# Autodesk Inventor assembly: POM_T5_02
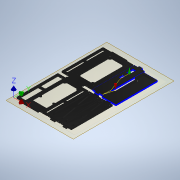
[picture p0: Inventor's stored thumbnail of the model, 180x180]
Saved by Autodesk Inventor 2020 (Build 240168000, 168)
## iProperties
Created: 2021-08-27
Part Number: POM_T5_02
Document SubType Name: Assembly
Designer: Masato
Author: Masato
## Documents named in this file (8)
- C:\Inventor\最新\OpenPlatform_ver3_0\Cam\POM_T5_02.iam
- C:\Inventor\最新\OpenPlatform_ver3_0\Cam\DisposableBoard.ipt
- C:\Inventor\最新\OpenPlatform_ver3_0\UpperBody\Cockpit\Cockpit_carrier_board_frame.ipt
- C:\Inventor\最新\OpenPlatform_ver3_0\UpperBody\Cockpit\Cockpit_circuit_board_frame.ipt
- C:\Inventor\最新\OpenPlatform_ver3_0\UpperBody\Cockpit\Cockpit_back_frame.ipt
- C:\Inventor\最新\OpenPlatform_ver3_0\UpperBody\Cockpit\Cockpit_battery_back_door.ipt
- C:\Inventor\最新\OpenPlatform_ver3_0\UpperBody\Cockpit\Cockpit_battery_bottom_frame.ipt
- C:\Inventor\最新\OpenPlatform_ver3_0\UpperBody\Cockpit\Cockpit_battery_front_frame.ipt
## Components (7 placed, 7 different names)
1. DisposableBoard:1 — メイト:2, メイト:1, フラッシュ:1, フラッシュ:2, メイト:4, メイト:6, メイト:7, メイト:8, メイト:9, フラッシュ:3, フラッシュ:4, フラッシュ:6, フラッシュ:7, メイト:17, フラッシュ:8
2. Cockpit_carrier_board_frame:1 — メイト:4, フラッシュ:3, フラッシュ:4, メイト:11, メイト:18
3. Cockpit_circuit_board_frame:1 — メイト:17, メイト:18, フラッシュ:8
4. Cockpit_back_frame:1 — メイト:9, メイト:12, メイト:16
5. Cockpit_battery_back_door:1 — メイト:8, メイト:15, メイト:16
6. Cockpit_battery_bottom_frame:1 — メイト:6, フラッシュ:6, メイト:11, メイト:12, メイト:14
7. Cockpit_battery_front_frame:1 — メイト:7, フラッシュ:7, メイト:14, メイト:15
## Relationships (21: Mate 14, Flush 7)
- メイト:2 [Mate]: DisposableBoard:1
- メイト:1 [Mate]: DisposableBoard:1
- フラッシュ:1 [Flush]: DisposableBoard:1
- フラッシュ:2 [Flush]: DisposableBoard:1
- メイト:4 [Mate]: DisposableBoard:1 ↔ Cockpit_carrier_board_frame:1
- メイト:6 [Mate]: DisposableBoard:1 ↔ Cockpit_battery_bottom_frame:1
- メイト:7 [Mate]: DisposableBoard:1 ↔ Cockpit_battery_front_frame:1
- メイト:8 [Mate]: DisposableBoard:1 ↔ Cockpit_battery_back_door:1
- メイト:9 [Mate]: DisposableBoard:1 ↔ Cockpit_back_frame:1
- フラッシュ:3 [Flush] (2.5 mm): DisposableBoard:1 ↔ Cockpit_carrier_board_frame:1
- フラッシュ:4 [Flush] (2.5 mm): DisposableBoard:1 ↔ Cockpit_carrier_board_frame:1
- フラッシュ:6 [Flush] (2.5 mm): DisposableBoard:1 ↔ Cockpit_battery_bottom_frame:1
- メイト:11 [Mate] (2.5 mm): Cockpit_carrier_board_frame:1 ↔ Cockpit_battery_bottom_frame:1
- メイト:12 [Mate] (2.5 mm): Cockpit_back_frame:1 ↔ Cockpit_battery_bottom_frame:1
- フラッシュ:7 [Flush] (2.5 mm): DisposableBoard:1 ↔ Cockpit_battery_front_frame:1
- メイト:14 [Mate] (2.5 mm): Cockpit_battery_bottom_frame:1 ↔ Cockpit_battery_front_frame:1
- メイト:15 [Mate] (2.5 mm): Cockpit_battery_back_door:1 ↔ Cockpit_battery_front_frame:1
- メイト:16 [Mate] (2.5 mm): Cockpit_back_frame:1 ↔ Cockpit_battery_back_door:1
- メイト:17 [Mate]: DisposableBoard:1 ↔ Cockpit_circuit_board_frame:1
- メイト:18 [Mate] (2.5 mm): Cockpit_carrier_board_frame:1 ↔ Cockpit_circuit_board_frame:1
- フラッシュ:8 [Flush] (2.5 mm): DisposableBoard:1 ↔ Cockpit_circuit_board_frame:1
